# Autodesk Inventor assembly: Grundplatte_test
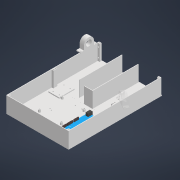
[picture p0: Inventor's stored thumbnail of the model, 180x180]
Saved by Autodesk Inventor 2021 (Build 250183000, 183)
## iProperties
Created: 2021-01-26
Part Number: Grundplatte_test
Document SubType Name: Assembly
Designer: Ctroi
Author: Ctroi
## Documents named in this file (9)
- E:\Projects\Rover\Grundplatte_test.iam
- E:\Projects\Rover\Grundplatte_hinten.ipt
- E:\Projects\Rover\Grundplatte_vorne.ipt
- E:\Projects\Rover\ArduinoMega.ipt
- E:\Projects\Rover\Relais.ipt
- E:\Projects\Rover\Kreuz_Halterung.ipt
- E:\Projects\Rover\Obenplatte_hinten.ipt
- E:\Projects\Rover\Obenplatte_vorne.ipt
- E:\Projects\Rover\Halterung_Differential_3.ipt
## Components (9 placed, 8 different names)
1. Grundplatte_hinten:1 — Passend:1, Passend:2, Passend:5, Passend:6, Passend:7, Passend:11, Passend:12, Passend:13, Passend:16
2. Grundplatte_vorne:1 — Passend:1, Passend:2, Passend:3, Passend:4, Passend:8, Passend:9, Passend:10, Passend:16
3. ArduinoMega:1 — Passend:3, Passend:4
4. Relais:1
5. Kreuz_Halterung:1 — Passend:5, Passend:6, Passend:7
6. Obenplatte_vorne:1 — Passend:8, Passend:9, Passend:10, Passend:15
7. Halterung_Differential_3:1 — Passend:14, Passend:15
8. Halterung_Differential_3:2
9. Obenplatte_hinten:1 — Passend:11, Passend:12, Passend:13, Passend:14
## Relationships (16: Mate 16)
- Passend:1 [Mate]: Grundplatte_hinten:1 ↔ Grundplatte_vorne:1
- Passend:2 [Mate]: Grundplatte_hinten:1 ↔ Grundplatte_vorne:1
- Passend:3 [Mate]: Grundplatte_vorne:1 ↔ ArduinoMega:1
- Passend:4 [Mate]: Grundplatte_vorne:1 ↔ ArduinoMega:1
- Passend:5 [Mate]: Grundplatte_hinten:1 ↔ Kreuz_Halterung:1
- Passend:6 [Mate]: Grundplatte_hinten:1 ↔ Kreuz_Halterung:1
- Passend:7 [Mate]: Grundplatte_hinten:1 ↔ Kreuz_Halterung:1
- Passend:8 [Mate]: Grundplatte_vorne:1 ↔ Obenplatte_vorne:1
- Passend:9 [Mate]: Grundplatte_vorne:1 ↔ Obenplatte_vorne:1
- Passend:10 [Mate]: Grundplatte_vorne:1 ↔ Obenplatte_vorne:1
- Passend:11 [Mate]: Grundplatte_hinten:1 ↔ Obenplatte_hinten:1
- Passend:12 [Mate]: Grundplatte_hinten:1 ↔ Obenplatte_hinten:1
- Passend:13 [Mate]: Grundplatte_hinten:1 ↔ Obenplatte_hinten:1
- Passend:14 [Mate]: Halterung_Differential_3:1 ↔ Obenplatte_hinten:1
- Passend:15 [Mate]: Obenplatte_vorne:1 ↔ Halterung_Differential_3:1
- Passend:16 [Mate]: Grundplatte_hinten:1 ↔ Grundplatte_vorne:1
